# Autodesk Inventor assembly: 细轴四方中间洞
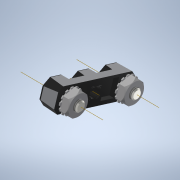
[picture p0: Inventor's stored thumbnail of the model, 180x180]
Saved by Autodesk Inventor 2020 (Build 240168000, 168)
## iProperties
Created: 2019-05-20
Part Number: 细轴四方中间洞
Material: 常规
Document SubType Name: Assembly
Designer: aresp
Mass: 17.9947 g
Surface Area: 29.0477 cm^2
Volume: 2.30445 cm^3
Density: 7.80868 g/cm^3
Author: aresp
## Documents named in this file (3)
- C:\towerTakeOverCad\ncrCadLib\细轴四方轴套套.iam
- C:\towerTakeOverCad\ncrCadLib\轴相关\细轴配套\细轴四方轴承.ipt
- C:\towerTakeOverCad\ncrCadLib\细轴四方轴套用的螺丝螺帽套.iam
## Components (3 placed, 2 different names)
1. 细轴四方轴承:1 — 配合:1, 配合:2, 配合:3
2. 细轴四方轴套用的螺丝螺帽套:1 [sub-assembly] — 表面齐平:1, 配合:1
3. 细轴四方轴套用的螺丝螺帽套:2 [sub-assembly] — 表面齐平:1, 配合:2, 配合:3
## Relationships (4: Mate 3, Flush 1)
- 表面齐平:1 [Flush]: 细轴四方轴套用的螺丝螺帽套:1 ↔ 细轴四方轴套用的螺丝螺帽套:2
- 配合:1 [Mate]: 细轴四方轴承:1 ↔ 细轴四方轴套用的螺丝螺帽套:1
- 配合:2 [Mate]: 细轴四方轴承:1 ↔ 细轴四方轴套用的螺丝螺帽套:2
- 配合:3 [Mate]: 细轴四方轴承:1 ↔ 细轴四方轴套用的螺丝螺帽套:2
